# Autodesk Inventor assembly: CableSupport-Knomi
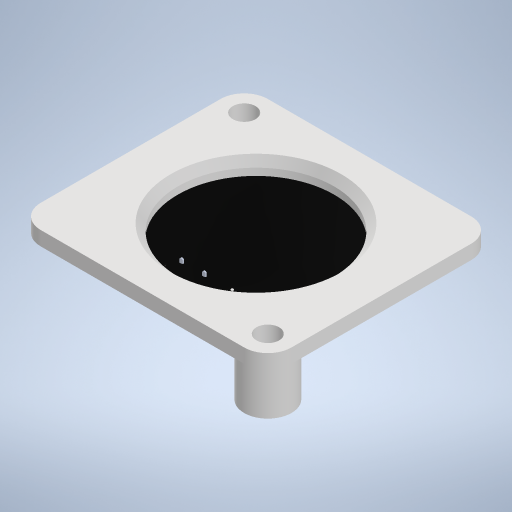
[picture p0: Inventor's stored thumbnail of the model, 512x512]
Saved by Autodesk Inventor 2023 (Build 270158000, 158)
## iProperties
Created: 2024-03-22
Part Number: CableSupport-Knomi
Document SubType Name: Assembly
Designer: incep
Author: incep
## Documents named in this file (3)
- C:\Users\incep\OneDrive\Desktop\3D Printer Stuff\Smart Orbiter V3 Design for Sigmax\CableSupport-Knomi.iam
- C:\Users\incep\OneDrive\Desktop\3D Printer Stuff\Smart Orbiter V3 Design for Sigmax\CableSupport-Knomi.ipt
- C:\Users\incep\OneDrive\Desktop\3D Printer Stuff\Smart Orbiter V3 Design for Sigmax\BIGTREETECH KNOMI v1.0.iam
## Components (2 placed, 2 different names)
1. CableSupport-Knomi:1 — Flush:1, Flush:2, Flush:3, Mate:1, Mate:2, Mate:3, Mate:4, Mate:5
2. BIGTREETECH KNOMI v1.0:1 [sub-assembly] — Mate:5, Angle:1
## Relationships (9: Mate 5, Flush 3, Angle 1)
- Flush:1: CableSupport-Knomi:1
- Flush:2: CableSupport-Knomi:1
- Flush:3: CableSupport-Knomi:1
- Mate:1: CableSupport-Knomi:1
- Mate:2: CableSupport-Knomi:1
- Mate:3: CableSupport-Knomi:1
- Mate:4: CableSupport-Knomi:1
- Mate:5: CableSupport-Knomi:1 ↔ BIGTREETECH KNOMI v1.0:1
- Angle:1 (0 deg): BIGTREETECH KNOMI v1.0:1
